# Autodesk Inventor assembly: square_alt_assem
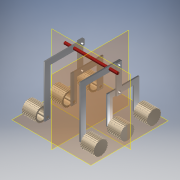
[picture p0: Inventor's stored thumbnail of the model, 180x180]
Saved by Autodesk Inventor 2018.1 (Build 221171000, 171)
## iProperties
Created: 2017-10-26
Part Number: square_alt_assem
Material: 一般
Document SubType Name: Assembly
Designer: Kakeru Yamashita
Author: Kakeru Yamashita
## Documents named in this file (10)
- C:\Users\Kakeru Yamashita\Documents\Inventor\forest_cad-master\Rocker_bogie_sim\square_alt_assem.iam
- C:\Users\Kakeru Yamashita\Documents\Inventor\forest_cad-master\Rocker_bogie_sim\bogie_square_alt.ipt
- C:\Users\Kakeru Yamashita\Documents\Inventor\forest_cad-master\Rocker_bogie_sim\tire.ipt
- C:\Users\Kakeru Yamashita\Documents\Inventor\forest_cad-master\Rocker_bogie_sim\rocker_bogie_plate.ipt
- C:\Users\Kakeru Yamashita\Documents\Inventor\forest_cad-master\Rocker_bogie_sim\rocker_alt.ipt
- C:\Users\Kakeru Yamashita\Documents\Inventor\forest_cad-master\Rocker_bogie_sim\sim_shaft.ipt
- C:\Users\Kakeru Yamashita\Documents\Inventor\forest_cad-master\Rocker_bogie_sim\bogie_square_alt_MIR.ipt
- C:\Users\Kakeru Yamashita\Documents\Inventor\forest_cad-master\Rocker_bogie_sim\tire_MIR1.ipt
- C:\Users\Kakeru Yamashita\Documents\Inventor\forest_cad-master\Rocker_bogie_sim\rocker_bogie_plate_MIR1.ipt
- C:\Users\Kakeru Yamashita\Documents\Inventor\forest_cad-master\Rocker_bogie_sim\rocker_alt_MIR.ipt
## Components (13 placed, 9 different names)
1. bogie_square_alt:1 — メイト:1, メイト:2, フラッシュ:2, メイト:6, メイト:7, フラッシュ:5
2. tire:1 — メイト:2, フラッシュ:1
3. tire:2 — メイト:1, フラッシュ:1, フラッシュ:2
4. tire:3 — メイト:8, フラッシュ:6
5. rocker_bogie_plate:1 — メイト:6, メイト:7, フラッシュ:5, メイト:9, メイト:10, フラッシュ:7
6. rocker_alt:1 — メイト:8, フラッシュ:6, メイト:9, メイト:10, フラッシュ:7, メイト:12, フラッシュ:10, フラッシュ:11, フラッシュ:12
7. sim_shaft:1 — フラッシュ:9, メイト:12, フラッシュ:10, フラッシュ:20
8. bogie_square_alt_MIR:1 — メイト:13, フラッシュ:13, メイト:14, フラッシュ:15, メイト:15, メイト:16
9. tire_MIR1:1 — メイト:13, フラッシュ:14
10. tire_MIR1:2 — フラッシュ:13, フラッシュ:14, メイト:14
11. tire_MIR1:3 — フラッシュ:19, メイト:19
12. rocker_bogie_plate_MIR1:1 — フラッシュ:15, メイト:15, メイト:16, フラッシュ:18, メイト:17, メイト:18
13. rocker_alt_MIR:1 — フラッシュ:16, フラッシュ:17, フラッシュ:18, メイト:17, メイト:18, フラッシュ:19, メイト:19, フラッシュ:20
## Relationships (32: Flush 17, Mate 15)
- メイト:1 [Mate]: bogie_square_alt:1 ↔ tire:2
- メイト:2 [Mate]: bogie_square_alt:1 ↔ tire:1
- フラッシュ:1 [Flush]: tire:1 ↔ tire:2
- フラッシュ:2 [Flush]: bogie_square_alt:1 ↔ tire:2
- メイト:6 [Mate]: bogie_square_alt:1 ↔ rocker_bogie_plate:1
- メイト:7 [Mate]: bogie_square_alt:1 ↔ rocker_bogie_plate:1
- フラッシュ:5 [Flush]: bogie_square_alt:1 ↔ rocker_bogie_plate:1
- メイト:8 [Mate]: tire:3 ↔ rocker_alt:1
- フラッシュ:6 [Flush]: tire:3 ↔ rocker_alt:1
- メイト:9 [Mate]: rocker_bogie_plate:1 ↔ rocker_alt:1
- メイト:10 [Mate]: rocker_bogie_plate:1 ↔ rocker_alt:1
- フラッシュ:7 [Flush]: rocker_bogie_plate:1 ↔ rocker_alt:1
- フラッシュ:9 [Flush] (100 mm): sim_shaft:1
- メイト:12 [Mate]: rocker_alt:1 ↔ sim_shaft:1
- フラッシュ:10 [Flush] (30 mm): rocker_alt:1 ↔ sim_shaft:1
- フラッシュ:11 [Flush] (110 mm): rocker_alt:1
- フラッシュ:12 [Flush] (210 mm): rocker_alt:1
- メイト:13 [Mate]: bogie_square_alt_MIR:1 ↔ tire_MIR1:1
- フラッシュ:13 [Flush]: bogie_square_alt_MIR:1 ↔ tire_MIR1:2
- フラッシュ:14 [Flush]: tire_MIR1:1 ↔ tire_MIR1:2
- メイト:14 [Mate]: bogie_square_alt_MIR:1 ↔ tire_MIR1:2
- フラッシュ:15 [Flush]: bogie_square_alt_MIR:1 ↔ rocker_bogie_plate_MIR1:1
- メイト:15 [Mate]: bogie_square_alt_MIR:1 ↔ rocker_bogie_plate_MIR1:1
- メイト:16 [Mate]: bogie_square_alt_MIR:1 ↔ rocker_bogie_plate_MIR1:1
- フラッシュ:16 [Flush] (210 mm): rocker_alt_MIR:1
- フラッシュ:17 [Flush] (110 mm): rocker_alt_MIR:1
- フラッシュ:18 [Flush]: rocker_bogie_plate_MIR1:1 ↔ rocker_alt_MIR:1
- メイト:17 [Mate]: rocker_bogie_plate_MIR1:1 ↔ rocker_alt_MIR:1
- メイト:18 [Mate]: rocker_bogie_plate_MIR1:1 ↔ rocker_alt_MIR:1
- フラッシュ:19 [Flush]: tire_MIR1:3 ↔ rocker_alt_MIR:1
- メイト:19 [Mate]: tire_MIR1:3 ↔ rocker_alt_MIR:1
- フラッシュ:20 [Flush] (30 mm): sim_shaft:1 ↔ rocker_alt_MIR:1
